# Autodesk Inventor assembly: Assembly1
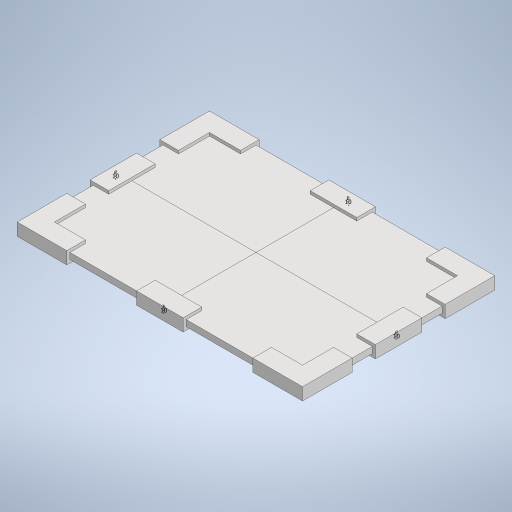
[picture p0: Inventor's stored thumbnail of the model, 512x512]
Saved by Autodesk Inventor 2024 (Build 280153000, 153)
## iProperties
Created: 2024-12-30
Part Number: Assembly1
Document SubType Name: Assembly
Designer: mtidd
Author: mtidd
## Documents named in this file (6)
- C:\Users\mtidd\OneDrive\Desktop\H2A\CAD\Trash Storage Unit\Assembly1.iam
- C:\Users\mtidd\OneDrive\Desktop\H2A\CAD\Trash Storage Unit\TSU_Baseplate_Female.ipt
- C:\Users\mtidd\OneDrive\Desktop\H2A\CAD\Trash Storage Unit\TSU_Baseplate_Male.ipt
- C:\Users\mtidd\OneDrive\Desktop\H2A\CAD\Trash Storage Unit\TSU_Baseplate_Male_Cut.ipt
- C:\Users\mtidd\OneDrive\Desktop\H2A\CAD\Trash Storage Unit\TSU_Middle_Clamp.ipt
- C:\Users\mtidd\OneDrive\Desktop\H2A\CAD\Trash Storage Unit\TSU_Corner_Clamp.ipt
## Components (12 placed, 5 different names)
1. TSU_Baseplate_Female:1 — Mate:1, Mate:2, Mate:10, Mate:12, Mate:18, Mate:19
2. TSU_Baseplate_Male:1 — Mate:1, Mate:2, Mate:3, Mate:4, Mate:9, Mate:13, Mate:15, Mate:20
3. TSU_Baseplate_Female:2 — Mate:3, Mate:4, Mate:5, Mate:6, Mate:7, Mate:14, Mate:16, Mate:21
4. TSU_Baseplate_Male_Cut:1 — Mate:5, Mate:6, Mate:8, Mate:11, Mate:17, Mate:22
5. TSU_Middle_Clamp:1 — Mate:7, Mate:13
6. TSU_Middle_Clamp:2 — Mate:9, Mate:12
7. TSU_Middle_Clamp:3 — Mate:10, Mate:11
8. TSU_Middle_Clamp:4 — Mate:8, Mate:14
9. TSU_Corner_Clamp:1 — Mate:15, Mate:20
10. TSU_Corner_Clamp:2 — Mate:18, Mate:19
11. TSU_Corner_Clamp:3 — Mate:17, Mate:22
12. TSU_Corner_Clamp:4 — Mate:16, Mate:21
## Relationships (22: Mate 22)
- Mate:1: TSU_Baseplate_Female:1 ↔ TSU_Baseplate_Male:1
- Mate:2: TSU_Baseplate_Female:1 ↔ TSU_Baseplate_Male:1
- Mate:3: TSU_Baseplate_Male:1 ↔ TSU_Baseplate_Female:2
- Mate:4: TSU_Baseplate_Male:1 ↔ TSU_Baseplate_Female:2
- Mate:5: TSU_Baseplate_Female:2 ↔ TSU_Baseplate_Male_Cut:1
- Mate:6: TSU_Baseplate_Female:2 ↔ TSU_Baseplate_Male_Cut:1
- Mate:7: TSU_Baseplate_Female:2 ↔ TSU_Middle_Clamp:1
- Mate:8: TSU_Baseplate_Male_Cut:1 ↔ TSU_Middle_Clamp:4
- Mate:9: TSU_Baseplate_Male:1 ↔ TSU_Middle_Clamp:2
- Mate:10: TSU_Baseplate_Female:1 ↔ TSU_Middle_Clamp:3
- Mate:11: TSU_Baseplate_Male_Cut:1 ↔ TSU_Middle_Clamp:3
- Mate:12: TSU_Baseplate_Female:1 ↔ TSU_Middle_Clamp:2
- Mate:13: TSU_Baseplate_Male:1 ↔ TSU_Middle_Clamp:1
- Mate:14: TSU_Baseplate_Female:2 ↔ TSU_Middle_Clamp:4
- Mate:15: TSU_Baseplate_Male:1 ↔ TSU_Corner_Clamp:1
- Mate:16: TSU_Baseplate_Female:2 ↔ TSU_Corner_Clamp:4
- Mate:17: TSU_Baseplate_Male_Cut:1 ↔ TSU_Corner_Clamp:3
- Mate:18: TSU_Baseplate_Female:1 ↔ TSU_Corner_Clamp:2
- Mate:19: TSU_Baseplate_Female:1 ↔ TSU_Corner_Clamp:2
- Mate:20: TSU_Baseplate_Male:1 ↔ TSU_Corner_Clamp:1
- Mate:21: TSU_Baseplate_Female:2 ↔ TSU_Corner_Clamp:4
- Mate:22: TSU_Baseplate_Male_Cut:1 ↔ TSU_Corner_Clamp:3
